# Autodesk Inventor assembly: Baugruppe1
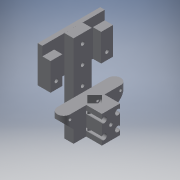
[picture p0: Inventor's stored thumbnail of the model, 180x180]
Saved by Autodesk Inventor 2019 (Build 230136000, 136)
## iProperties
Created: 2021-06-02
Part Number: Baugruppe1
Material: Generisch
Document SubType Name: Assembly
Designer: Bergi
Author: Bergi
## Documents named in this file (4)
- C:\Users\Bergi\Desktop\3D Sketches\Bleistift_Plotter\V3\Baugruppe1.iam
- C:\Users\Bergi\Desktop\3D Sketches\Bleistift_Plotter\V3\Schlitten_neu.ipt
- C:\Users\Bergi\Desktop\3D Sketches\Bleistift_Plotter\V3\Backplate.ipt
- C:\Users\Bergi\Desktop\3D Sketches\Bleistift_Plotter\V3\Linear_rail.ipt
## Components (3 placed, 3 different names)
1. Schlitten_neu:1 — Passend:1, Passend:2
2. Backplate:1 — Passend:5, Passend:8, Passend:9
3. Linear_rail:1 — Passend:1, Passend:2, Passend:5, Passend:8, Passend:9
## Relationships (5: Mate 5)
- Passend:1 [Mate]: Schlitten_neu:1 ↔ Linear_rail:1
- Passend:2 [Mate]: Schlitten_neu:1 ↔ Linear_rail:1
- Passend:5 [Mate]: Backplate:1 ↔ Linear_rail:1
- Passend:8 [Mate]: Backplate:1 ↔ Linear_rail:1
- Passend:9 [Mate]: Backplate:1 ↔ Linear_rail:1
